# Autodesk Inventor assembly: Manipulator
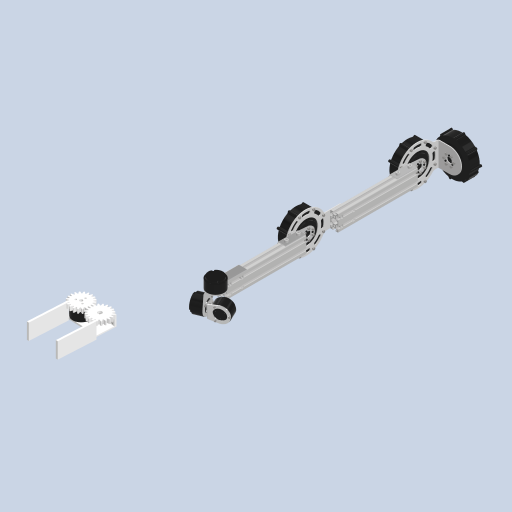
[picture p0: Inventor's stored thumbnail of the model, 512x512]
Saved by Autodesk Inventor 2023 (Build 270158000, 158)
## iProperties
Created: 2024-11-08
Part Number: Manipulator
Document SubType Name: Assembly
Designer: kiyo
Author: kiyo
## Documents named in this file (23)
- D:\GitHub\inventor\syu-si\OfficeRobot\Manipulator\Manipulator.iam
- D:\GitHub\inventor\syu-si\OfficeRobot\ReadyMade\Steadywin\GIM8108-8.iam
- D:\GitHub\inventor\syu-si\OfficeRobot\Manipulator\sholder-roll-bracket.ipt
- D:\GitHub\inventor\syu-si\OfficeRobot\Manipulator\elbow-pitch-bracket.ipt
- D:\GitHub\inventor\syu-si\OfficeRobot\Manipulator\Hand.iam
- D:\GitHub\inventor\syu-si\OfficeRobot\ReadyMade\Screw\M3_7mm.ipt
- D:\GitHub\inventor\syu-si\OfficeRobot\ReadyMade\Screw\M3_6mm.ipt
- D:\GitHub\inventor\syu-si\OfficeRobot\ReadyMade\Screw\M2-5_4mm.ipt
- D:\GitHub\inventor\syu-si\OfficeRobot\ReadyMade\Screw\M2-5_5mm.ipt
- D:\GitHub\inventor\syu-si\OfficeRobot\ReadyMade\Screw\M2-5_7mm.ipt
- D:\GitHub\inventor\syu-si\OfficeRobot\ReadyMade\Screw\SCB5-22.ipt
- D:\GitHub\inventor\syu-si\OfficeRobot\ReadyMade\Screw\HNTP5-5.ipt
- D:\GitHub\inventor\syu-si\OfficeRobot\Manipulator\pitch_plate_40mm.ipt
- D:\GitHub\inventor\syu-si\OfficeRobot\ReadyMade\Steadywin\GIM3505-8_with-driver.ipt
- D:\GitHub\inventor\syu-si\OfficeRobot\Manipulator\wrist_roll_plate.ipt
- D:\GitHub\inventor\syu-si\OfficeRobot\Manipulator\wrist-pitch-plate.ipt
- D:\GitHub\inventor\syu-si\OfficeRobot\Manipulator\wrist-yaw-plate.ipt
- D:\GitHub\inventor\syu-si\OfficeRobot\ReadyMade\Screw\M2-5_6mm.ipt
- D:\GitHub\inventor\syu-si\OfficeRobot\ReadyMade\Screw\FWSJJ-D5-V2_6-T4.ipt
- D:\GitHub\inventor\syu-si\OfficeRobot\ReadyMade\Screw\M2-5_9mm.ipt
- D:\GitHub\inventor\syu-si\OfficeRobot\ReadyMade\Aluminum-frame\HFS5-2040-200-AV160-BV190-Z5-YA10-YB40.ipt
- D:\GitHub\inventor\syu-si\OfficeRobot\ReadyMade\Screw\SCB5-46.ipt
- D:\GitHub\inventor\syu-si\OfficeRobot\ReadyMade\Screw\SLBNR5.ipt
## Components (100 placed, 22 different names)
1. elbow-pitch-bracket:1 — 挿入:172, 挿入:173, 挿入:174, 挿入:175, 挿入:176, 挿入:177, 挿入:178, 挿入:179, 挿入:180, 挿入:181, 挿入:234, 挿入:235, 挿入:256, 挿入:257
2. sholder-roll-bracket:1 — 挿入:1, 挿入:2, 挿入:3, 肩ヨー, 挿入:94, 挿入:95, 挿入:96, 挿入:97, 挿入:98, 挿入:99, 挿入:100, 挿入:101, 挿入:102, 挿入:103, 挿入:104, 挿入:105, 挿入:106, 挿入:107
3. pitch_plate_40mm:1 — 挿入:165, 挿入:182, 挿入:183, 挿入:184, 挿入:185, 挿入:186, 挿入:187, 挿入:232, 挿入:233, 角度:7, 挿入:250, 挿入:251, 挿入:254, 挿入:255
4. pitch_plate_40mm:2 — 挿入:190, 挿入:191, 挿入:192, 挿入:193, 挿入:194, 挿入:195, 挿入:196, 角度:8, 挿入:236, 挿入:237, 挿入:248, 挿入:249, 挿入:252, 挿入:253
5. wrist_roll_plate:1 — 挿入:214, 挿入:215, 挿入:216, 挿入:220, 挿入:224, 挿入:225, 挿入:226, 挿入:227, 挿入:228, 挿入:229, 挿入:230, 挿入:231
6. wrist-pitch-plate:1 — 挿入:208, 挿入:209, 挿入:210, 挿入:211, 挿入:212, 挿入:213, 挿入:217, 挿入:218, 挿入:219, 挿入:220, 挿入:221, 挿入:222, 挿入:223
7. wrist-yaw-plate:1 — 挿入:203, 挿入:204, 挿入:205, 挿入:206, 挿入:207, 挿入:211, 挿入:238, 挿入:239, 挿入:258, 挿入:259
8. HFS5-2040-200-AV160-BV190-Z5-YA10-YB40:1 — 挿入:232, 挿入:233, 挿入:234, 挿入:235, 挿入:246, 挿入:247
9. HFS5-2040-200-AV160-BV190-Z5-YA10-YB40:2 — 挿入:236, 挿入:237, 挿入:238, 挿入:239, 挿入:244, 挿入:245
10. Hand:1 [sub-assembly] — ハンド, 挿入:128, 挿入:129, 挿入:130, 挿入:131, 挿入:138, 挿入:139, 挿入:140, 挿入:141, 挿入:142, 挿入:143, 挿入:144
11. SCB5-22:1 — 挿入:247
12. SCB5-22:2 — 挿入:246
13. SCB5-22:3 — 挿入:244
14. SCB5-22:4 — 挿入:245
15. SCB5-46:1 — 挿入:250
16. SCB5-46:2 — 挿入:251
17. SCB5-46:3 — 挿入:248
18. SCB5-46:4 — 挿入:249
19. SLBNR5:1 — 挿入:255
20. SLBNR5:2 — 挿入:254
21. SLBNR5:3 — 挿入:252
22. SLBNR5:4 — 挿入:253
23. SLBNR5:5 — 挿入:256
24. SLBNR5:6 — 挿入:257
25. SLBNR5:7 — 挿入:258
26. SLBNR5:8 — 挿入:259
27. M3_6mm:1 — 挿入:183
28. M3_6mm:2 — 挿入:186
29. M3_6mm:3 — 挿入:187
30. M3_6mm:4 — 挿入:184
31. M3_6mm:5 — 挿入:185
32. M3_6mm:6 — 挿入:182
33. M3_6mm:7 — 挿入:192
34. M3_6mm:8 — 挿入:191
35. M3_6mm:9 — 挿入:196
36. M3_6mm:10 — 挿入:195
37. M3_6mm:11 — 挿入:194
38. M3_6mm:12 — 挿入:193
39. M3_6mm:13 — 挿入:107
40. M3_6mm:14 — 挿入:106
41. M3_6mm:15 — 挿入:105
42. M3_6mm:16 — 挿入:102
43. M3_6mm:17 — 挿入:103
44. M3_6mm:18 — 挿入:104
45. M3_7mm:1 — 挿入:144
46. M3_7mm:2 — 挿入:101
47. M3_7mm:3 — 挿入:100
48. M3_7mm:4 — 挿入:99
49. M3_7mm:5 — 挿入:97
50. M3_7mm:6 — 挿入:98
51. M3_7mm:7 — 挿入:96
52. M3_7mm:8 — 挿入:95
53. M3_7mm:9 — 挿入:94
54. M3_7mm:10 — 挿入:174
55. M3_7mm:11 — 挿入:179
56. M3_7mm:12 — 挿入:176
57. M3_7mm:13 — 挿入:173
58. M3_7mm:14 — 挿入:172
59. M3_7mm:15 — 挿入:175
60. M3_7mm:16 — 挿入:178
61. M3_7mm:17 — 挿入:177
62. M2-5_4mm:9 — 挿入:129
63. M2-5_4mm:10 — 挿入:130
64. M2-5_4mm:11 — 挿入:131
65. M2-5_4mm:12 — 挿入:128
66. M2-5_5mm:7 — 挿入:138
67. M2-5_5mm:8 — 挿入:139
68. M2-5_5mm:9 — 挿入:140
69. M2-5_6mm:1 — 挿入:205
70. M2-5_6mm:2 — 挿入:207
71. M2-5_6mm:3 — 挿入:206
72. M2-5_6mm:7 — 挿入:229
73. M2-5_6mm:8 — 挿入:230
74. M2-5_6mm:9 — 挿入:231
75. M2-5_6mm:4 — 挿入:217
76. M2-5_6mm:5 — 挿入:218
77. M2-5_6mm:6 — 挿入:219
78. M2-5_7mm:1 — 挿入:141
79. M2-5_7mm:2 — 挿入:142
80. M2-5_7mm:3 — 挿入:143
81. M2-5_9mm:1 — 挿入:221
82. M2-5_9mm:2 — 挿入:222
83. M2-5_9mm:3 — 挿入:223
84. M2-5_9mm:4 — 挿入:225
85. M2-5_9mm:5 — 挿入:226
86. M2-5_9mm:6 — 挿入:224
87. FWSJJ-D5-V2_6-T4:4 — 挿入:214
88. FWSJJ-D5-V2_6-T4:5 — 挿入:216
89. FWSJJ-D5-V2_6-T4:6 — 挿入:215
90. FWSJJ-D5-V2_6-T4:1 — 挿入:210
91. FWSJJ-D5-V2_6-T4:2 — 挿入:209
92. FWSJJ-D5-V2_6-T4:3 — 挿入:208
93. HNTP5-5:7
94. HNTP5-5:8
95. GIM3505-8_with-driver:1 — 挿入:203, 挿入:204
96. GIM3505-8_with-driver:3 — 挿入:227, 挿入:228
97. GIM3505-8_with-driver:4 — 挿入:212, 挿入:213
98. GIM8108-8:1 [sub-assembly] — 挿入:1
99. GIM8108-8:2 [sub-assembly] — 挿入:2, 挿入:3, 挿入:165
100. GIM8108-8:3 [sub-assembly] — 挿入:180, 挿入:181, 挿入:190
## Relationships (109: Insert 105, Angle 4)
- 挿入:1 [Insert]: sholder-roll-bracket:1 ↔ GIM8108-8:1
- 挿入:2 [Insert]: sholder-roll-bracket:1 ↔ GIM8108-8:2
- 挿入:3 [Insert]: sholder-roll-bracket:1 ↔ GIM8108-8:2
- 肩ヨー [Angle] (0 deg): sholder-roll-bracket:1
- ハンド [Angle] (0 deg): Hand:1
- 挿入:94 [Insert]: sholder-roll-bracket:1 ↔ M3_7mm:9
- 挿入:95 [Insert]: sholder-roll-bracket:1 ↔ M3_7mm:8
- 挿入:96 [Insert]: sholder-roll-bracket:1 ↔ M3_7mm:7
- 挿入:97 [Insert]: sholder-roll-bracket:1 ↔ M3_7mm:5
- 挿入:98 [Insert]: sholder-roll-bracket:1 ↔ M3_7mm:6
- 挿入:99 [Insert]: sholder-roll-bracket:1 ↔ M3_7mm:4
- 挿入:100 [Insert]: sholder-roll-bracket:1 ↔ M3_7mm:3
- 挿入:101 [Insert]: sholder-roll-bracket:1 ↔ M3_7mm:2
- 挿入:102 [Insert]: sholder-roll-bracket:1 ↔ M3_6mm:16
- 挿入:103 [Insert]: sholder-roll-bracket:1 ↔ M3_6mm:17
- 挿入:104 [Insert]: sholder-roll-bracket:1 ↔ M3_6mm:18
- 挿入:105 [Insert]: sholder-roll-bracket:1 ↔ M3_6mm:15
- 挿入:106 [Insert]: sholder-roll-bracket:1 ↔ M3_6mm:14
- 挿入:107 [Insert]: sholder-roll-bracket:1 ↔ M3_6mm:13
- 挿入:128 [Insert]: Hand:1 ↔ M2-5_4mm:12
- 挿入:129 [Insert]: Hand:1 ↔ M2-5_4mm:9
- 挿入:130 [Insert]: Hand:1 ↔ M2-5_4mm:10
- 挿入:131 [Insert]: Hand:1 ↔ M2-5_4mm:11
- 挿入:138 [Insert]: Hand:1 ↔ M2-5_5mm:7
- 挿入:139 [Insert]: Hand:1 ↔ M2-5_5mm:8
- 挿入:140 [Insert]: Hand:1 ↔ M2-5_5mm:9
- 挿入:141 [Insert]: Hand:1 ↔ M2-5_7mm:1
- 挿入:142 [Insert]: Hand:1 ↔ M2-5_7mm:2
- 挿入:143 [Insert]: Hand:1 ↔ M2-5_7mm:3
- 挿入:144 [Insert]: Hand:1 ↔ M3_7mm:1
- 挿入:165 [Insert]: pitch_plate_40mm:1 ↔ GIM8108-8:2
- 挿入:172 [Insert]: elbow-pitch-bracket:1 ↔ M3_7mm:14
- 挿入:173 [Insert]: elbow-pitch-bracket:1 ↔ M3_7mm:13
- 挿入:174 [Insert]: elbow-pitch-bracket:1 ↔ M3_7mm:10
- 挿入:175 [Insert]: elbow-pitch-bracket:1 ↔ M3_7mm:15
- 挿入:176 [Insert]: elbow-pitch-bracket:1 ↔ M3_7mm:12
- 挿入:177 [Insert]: elbow-pitch-bracket:1 ↔ M3_7mm:17
- 挿入:178 [Insert]: elbow-pitch-bracket:1 ↔ M3_7mm:16
- 挿入:179 [Insert]: elbow-pitch-bracket:1 ↔ M3_7mm:11
- 挿入:180 [Insert]: elbow-pitch-bracket:1 ↔ GIM8108-8:3
- 挿入:181 [Insert]: elbow-pitch-bracket:1 ↔ GIM8108-8:3
- 挿入:182 [Insert]: pitch_plate_40mm:1 ↔ M3_6mm:6
- 挿入:183 [Insert]: pitch_plate_40mm:1 ↔ M3_6mm:1
- 挿入:184 [Insert]: pitch_plate_40mm:1 ↔ M3_6mm:4
- 挿入:185 [Insert]: pitch_plate_40mm:1 ↔ M3_6mm:5
- 挿入:186 [Insert]: pitch_plate_40mm:1 ↔ M3_6mm:2
- 挿入:187 [Insert]: pitch_plate_40mm:1 ↔ M3_6mm:3
- 挿入:190 [Insert]: pitch_plate_40mm:2 ↔ GIM8108-8:3
- 挿入:191 [Insert]: pitch_plate_40mm:2 ↔ M3_6mm:8
- 挿入:192 [Insert]: pitch_plate_40mm:2 ↔ M3_6mm:7
- 挿入:193 [Insert]: pitch_plate_40mm:2 ↔ M3_6mm:12
- 挿入:194 [Insert]: pitch_plate_40mm:2 ↔ M3_6mm:11
- 挿入:195 [Insert]: pitch_plate_40mm:2 ↔ M3_6mm:10
- 挿入:196 [Insert]: pitch_plate_40mm:2 ↔ M3_6mm:9
- 挿入:203 [Insert]: wrist-yaw-plate:1 ↔ GIM3505-8_with-driver:1
- 挿入:204 [Insert]: wrist-yaw-plate:1 ↔ GIM3505-8_with-driver:1
- 挿入:205 [Insert]: wrist-yaw-plate:1 ↔ M2-5_6mm:1
- 挿入:206 [Insert]: wrist-yaw-plate:1 ↔ M2-5_6mm:3
- 挿入:207 [Insert]: wrist-yaw-plate:1 ↔ M2-5_6mm:2
- 挿入:208 [Insert]: wrist-pitch-plate:1 ↔ FWSJJ-D5-V2_6-T4:3
- 挿入:209 [Insert]: wrist-pitch-plate:1 ↔ FWSJJ-D5-V2_6-T4:2
- 挿入:210 [Insert]: wrist-pitch-plate:1 ↔ FWSJJ-D5-V2_6-T4:1
- 挿入:211 [Insert] (3 mm): wrist-pitch-plate:1 ↔ wrist-yaw-plate:1
- 挿入:212 [Insert]: wrist-pitch-plate:1 ↔ GIM3505-8_with-driver:4
- 挿入:213 [Insert]: wrist-pitch-plate:1 ↔ GIM3505-8_with-driver:4
- 挿入:214 [Insert]: wrist_roll_plate:1 ↔ FWSJJ-D5-V2_6-T4:4
- 挿入:215 [Insert]: wrist_roll_plate:1 ↔ FWSJJ-D5-V2_6-T4:6
- 挿入:216 [Insert]: wrist_roll_plate:1 ↔ FWSJJ-D5-V2_6-T4:5
- 挿入:217 [Insert]: wrist-pitch-plate:1 ↔ M2-5_6mm:4
- 挿入:218 [Insert]: wrist-pitch-plate:1 ↔ M2-5_6mm:5
- 挿入:219 [Insert]: wrist-pitch-plate:1 ↔ M2-5_6mm:6
- 挿入:220 [Insert] (3 mm): wrist_roll_plate:1 ↔ wrist-pitch-plate:1
- 挿入:221 [Insert]: wrist-pitch-plate:1 ↔ M2-5_9mm:1
- 挿入:222 [Insert]: wrist-pitch-plate:1 ↔ M2-5_9mm:2
- 挿入:223 [Insert]: wrist-pitch-plate:1 ↔ M2-5_9mm:3
- 挿入:224 [Insert]: wrist_roll_plate:1 ↔ M2-5_9mm:6
- 挿入:225 [Insert]: wrist_roll_plate:1 ↔ M2-5_9mm:4
- 挿入:226 [Insert]: wrist_roll_plate:1 ↔ M2-5_9mm:5
- 挿入:227 [Insert]: wrist_roll_plate:1 ↔ GIM3505-8_with-driver:3
- 挿入:228 [Insert]: wrist_roll_plate:1 ↔ GIM3505-8_with-driver:3
- 挿入:229 [Insert]: wrist_roll_plate:1 ↔ M2-5_6mm:7
- 挿入:230 [Insert]: wrist_roll_plate:1 ↔ M2-5_6mm:8
- 挿入:231 [Insert]: wrist_roll_plate:1 ↔ M2-5_6mm:9
- 挿入:232 [Insert]: pitch_plate_40mm:1 ↔ HFS5-2040-200-AV160-BV190-Z5-YA10-YB40:1
- 挿入:233 [Insert]: pitch_plate_40mm:1 ↔ HFS5-2040-200-AV160-BV190-Z5-YA10-YB40:1
- 挿入:234 [Insert] (6 mm): elbow-pitch-bracket:1 ↔ HFS5-2040-200-AV160-BV190-Z5-YA10-YB40:1
- 挿入:235 [Insert] (6 mm): elbow-pitch-bracket:1 ↔ HFS5-2040-200-AV160-BV190-Z5-YA10-YB40:1
- 角度:7 [Angle] (0 deg): pitch_plate_40mm:1
- 角度:8 [Angle] (0 deg): pitch_plate_40mm:2
- 挿入:236 [Insert]: pitch_plate_40mm:2 ↔ HFS5-2040-200-AV160-BV190-Z5-YA10-YB40:2
- 挿入:237 [Insert]: pitch_plate_40mm:2 ↔ HFS5-2040-200-AV160-BV190-Z5-YA10-YB40:2
- 挿入:238 [Insert] (6 mm): wrist-yaw-plate:1 ↔ HFS5-2040-200-AV160-BV190-Z5-YA10-YB40:2
- 挿入:239 [Insert] (6 mm): wrist-yaw-plate:1 ↔ HFS5-2040-200-AV160-BV190-Z5-YA10-YB40:2
- 挿入:244 [Insert]: HFS5-2040-200-AV160-BV190-Z5-YA10-YB40:2 ↔ SCB5-22:3
- 挿入:245 [Insert]: HFS5-2040-200-AV160-BV190-Z5-YA10-YB40:2 ↔ SCB5-22:4
- 挿入:246 [Insert]: HFS5-2040-200-AV160-BV190-Z5-YA10-YB40:1 ↔ SCB5-22:2
- 挿入:247 [Insert]: HFS5-2040-200-AV160-BV190-Z5-YA10-YB40:1 ↔ SCB5-22:1
- 挿入:248 [Insert]: pitch_plate_40mm:2 ↔ SCB5-46:3
- 挿入:249 [Insert]: pitch_plate_40mm:2 ↔ SCB5-46:4
- 挿入:250 [Insert]: pitch_plate_40mm:1 ↔ SCB5-46:1
- 挿入:251 [Insert]: pitch_plate_40mm:1 ↔ SCB5-46:2
- 挿入:252 [Insert]: pitch_plate_40mm:2 ↔ SLBNR5:3
- 挿入:253 [Insert]: pitch_plate_40mm:2 ↔ SLBNR5:4
- 挿入:254 [Insert]: pitch_plate_40mm:1 ↔ SLBNR5:2
- 挿入:255 [Insert]: pitch_plate_40mm:1 ↔ SLBNR5:1
- 挿入:256 [Insert]: elbow-pitch-bracket:1 ↔ SLBNR5:5
- 挿入:257 [Insert]: elbow-pitch-bracket:1 ↔ SLBNR5:6
- 挿入:258 [Insert]: wrist-yaw-plate:1 ↔ SLBNR5:7
- 挿入:259 [Insert]: wrist-yaw-plate:1 ↔ SLBNR5:8
